# Autodesk Inventor assembly: HTPB14S2M040-K-P3
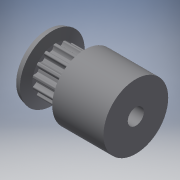
[picture p0: Inventor's stored thumbnail of the model, 180x180]
Saved by Autodesk Inventor 2019 (Build 230136000, 136)
## iProperties
Category: PARTsolutions
Company: MISUMI
Created: 2023-12-23
Part Number: HTPB14S2M040-K-P3
Catalog Web Link: www.cadenas.de
Description: HTPA_ _S2M040, HTPA_ _S2M060, HTPA_ _S2M100, HTPB_ _S2M040, HTPB_ _S2M060, HTPB_ _S2M100, HTPK_ _S2M040, HTPK_ _S2M060, HTPK_ _S2M100, HTPN_ _S2M040, HTPN_ _S2M060, HTPN_ _S2M100, HTPT_ _S2M040, HTPT_ _S2M060, HTPM_ _S2M040, HTPM_ _S2M060, HTPP_ _S2M040, HTPP_ _S2M060, HTPS_ _S2M040, HTPS_ _S2M060, HTPS_ _S2M100-High Torque Timing Pulleys S2M Type
Vendor: MISUMI
Document SubType Name: Assembly
Designer: psAdmin
Manufacturer: MISUMI
Mass: 1.35006 g
Surface Area: 12.4331 cm^2
Volume: 1.35006 cm^3
Density: 1 g/cm^3
Title: HTPB14S2M040-K-P3
Author: Cadenas PARTsolutions
Comments: High Torque Timing Pulleys S2M Type
PSOL_IDENT_0: {$CADENAS_DATA/23d-libs/misumi/metric/51_timing_pulleys/htpm_s2m_asmtab.prj},744 {VTYP=3D},{STYP=ASS
PSOL_IDENT_1: TAB},{NB=HTPB14S2M040-K-P3},{LINA=HTPB14S2M040-K-P3},{NN=HTPA_ _S2M040, HTPA_ _S2M060, HTPA_ _S2M100
PSOL_IDENT_2: , HTPB_ _S2M040, HTPB_ _S2M060, HTPB_ _S2M100, HTPK_ _S2M040, HTPK_ _S2M060, HTPK_ _S2M100, HTPN_ _S
PSOL_IDENT_3: 2M040, HTPN_ _S2M060, HTPN_ _S2M100, HTPT_ _S2M040, HTPT_ _S2M060, HTPM_ _S2M040, HTPM_ _S2M060, HTP
PSOL_IDENT_4: P_ _S2M040, HTPP_ _S2M060, HTPS_ _S2M040, HTPS_ _S2M060, HTPS_ _S2M100},{DATE=13.01.2023 00:39:47},{
PSOL_IDENT_5: GEOMDATE=09.12.2022 07:33:44},{VERSION=},{LINEID=10},{WBVAR=MATP,ST,TNW,PS,SBS,DD,Z,J,Q,R,S,T,ALT1,A
PSOL_IDENT_6: LT2,M,QSC,QFC,QTC,ALT3,K,KSC,KFC,KTC,ALT4,ZM,ZSC,ZFC,ZTC,ALT5,ALT6,ALT7,FC,ALT8,SRG,ALT9,BTC,TL,ALT1
PSOL_IDENT_7: 0,TPC,ALT11,BC,ALT12,SLH,ALT13,BN},{WBNUMERIC=DD,Z,J,Q,R,S,T,QSC,QFC,QTC,K,KSC,KFC,KTC,ZSC,ZFC,ZTC,F
PSOL_IDENT_8: C,SRG,BTC,TL,BC,SLH,BN}  {NB=HTPB14S2M040-K-P3},{LINA=HTPB14S2M040-K-P3},{KT=DUMMY},{PN=HTPB14S2M040
PSOL_IDENT_9: -K-P3},{TYPE=HTPB},{MATP=A2017},{MATPALG= 'A2017','Aluminum Alloy 2000 series','S45CE','1045 Carbon
PSOL_IDENT_10: Steel Equivalent','SUS304','304 Stainless Steel' },{ST=BA},{STALG= 'CA' , 'Clear Anodize', 'BA','Bla
PSOL_IDENT_11: ck Anodize','HAT','Hard Clear Anodize' , 'ENP' , 'Electroless Nickel Plating' },{NT=14},{TNW=S2M040}
PSOL_IDENT_12: ,{TNWALG= 'S2M040', 'S2M060','S2M100' },{BW=4},{PS=K},{PSALG='A','K'},{SBS=P},{SBSALG='H','Round Hol
PSOL_IDENT_13: e','P','Round Hole + Tap'},{SHSA= 'H','Round Hole' },{SHSB='H','Round Hole','P','Round Hole + Tap','
PSOL_IDENT_14: N','New JIS Keywayed Bore + Tap (Standard)','NK','New JIS Keywayed Bore + Tap (width 4.0mm, height 1
PSOL_IDENT_15: .8mm)','C','Old JIS Keywayed Bore + Tap','V','Stepped Hole','F','Stepped Hole (Counterbore holes on
PSOL_IDENT_16: the boss side)' },{SHSK='H','Round Hole','P','Round Hole + Tap'},{SBSPN=-P3},{DD=3.00},{DDALG=[3:4/1
PSOL_IDENT_17: ]},{DDHA=0},{DDHBK=[3:4/1]},{DDPA=0},{DDPBK=[3:4/1]},{DDNA=0},{DDNBK=0},{DDNK=0},{DDCA=0},{DDCBK=0},
PSOL_IDENT_18: {DDVA=0},{DDVF=0},{DDY=0},{DDWB=0},{Z=0},{ZALG=[0]},{ZQRMIN=5},{ZAMAX=0},{ZBMAX=0},{DDZ=3},{J=0.0},{
PSOL_IDENT_19: JALG=[0]},{JMAX=0},{JMIN=2},{JPN=},{QRMAX=0},{QRMIN=5},{WBRMAX=-2.00},{WBQMIN=7},{Q=0},{QALG=[0]},{Q
PSOL_IDENT_20: PN=},{R=0},{RALG=[0]},{S=0.0},{SALG=[0]},{SPN=},{SMAX=3},{T=0.0},{TALG=[0]},{TPN=},{TMAX=6},{A=5},{W=
PSOL_IDENT_21: 9},{L=17},{PD=8.91},{OD=8.40},{D=12},{DALG=12},{DE=12},{F=12},{E=6},{BBK=0.000},{TTK=0.0},{TT=1},{WL=
PSOL_IDENT_22: 17.000},{ALT1=},{ALT1ALG= '','w/o KC90 (Set Screw Angle)','KC90','with KC90 (Set Screw Angle)' },{AN
PSOL_IDENT_23: G=120.000},{ALT1PN=},{ALT2=},{ALT2ALG= '','Not applicable' },{M=N/A},{MALG= 'N/A' },{MFTALG= 'N/A' }
PSOL_IDENT_24: ,{MSALG= 'N/A' },{M3D=0.000},{KDML=0},{ML=0},{MUL=0},{PITCH=0},{QSC=0.0},{QSCALG=0},{QFC=0.0},{QFCAL
PSOL_IDENT_25: G=0},{QTC=0.0},{QTCALG=0},{QPCDMIN=0},{QPCDMINALG=0},{QPCDMAX=8},{ALT2PN=},{ALT3=},{ALT3ALG= '','Not
PSOL_IDENT_26: applicable' },{K=0.0},{KALG=0},{KMIN=4},{KFTMAX=0.0},{KSMAX=0.0},{KSC=0.0},{KSCALG=0},{KFC=0.0},{KF
PSOL_IDENT_27: CALG=0},{KTC=0.0},{KTCALG=0},{KPCDMIN=7},{KPCDMINALG=7},{KPCDMAX=0},{KSCMIN=7.0},{KSCMINALG=7},{ALT3
PSOL_IDENT_28: PN=},{ALT4=},{ALT4ALG= '','Not applicable' },{ALT4MIN=13.5},{ALT4MAX=-4.5},{ZM=N/A},{ZMALG= 'N/A' },
PSOL_IDENT_29: {ZMSALG= 'N/A' },{ZMFTALG= 'N/A' },{ZMDD1=0.0},{ZMDD2=0.0},{ZMHH=0.0},{ZSC=0.0},{ZSCALG=[0]},{ZFC=0.
PSOL_IDENT_30: 0},{ZFCALG=[0]},{ZTC=0.0},{ZTCALG=[0]},{ZPCDMIN=0},{ZPCDMINALG=0},{ZPCDMAX=2},{ALT4PN=},{ALT5=},{ALT
PSOL_IDENT_31: 5ALG= '','Flange Attached','NFC','with NFC (Flange not Attached)' },{ALT5PN=},{ALT6=},{ALT6ALG= '','
PSOL_IDENT_32: Not applicable' },{ALT6PN=},{ALT7=},{ALT7ALG= '','w/o FC (Flange Cut)','FC','with FC (Flange Cut)' }
PSOL_IDENT_33: ,{FC=0.0},{FCALG=0},{FCMIN=9.5},{FCMAX=10.0},{ALT7PN=},{ALT8=},{ALT8ALG= '','Not applicable' },{ALT8
PSOL_IDENT_34: ALGALG=8},{ALT8DD2=0},{ALT8MM=0},{ALT8NN=0},{QC=0},{KC=0},{ZC=0},{SRG=0.0},{SRGALG=[0]},{SRGMAX=0},{
PSOL_IDENT_35: DD2=0.0},{MM=0.00},{NN=0.00},{ALT8PN=},{ALT9ALG= '','Not applicable' },{ALT9=},{BTC9=4},{TL9=1},{BTC=
PSOL_IDENT_36: 0},{BTCALG=[0]},{TL=0.0},{TLALG=[0]},{TLMIN=1.000},{TLMAX=-9.500},{BTCL=0},{BTCD=0},{BTCDALG=6.000},
PSOL_IDENT_37: {ALT9PN=},{WLBCTL=17},{ALT10=},{ALT10ALG= '','w/o TPC (Tapped Hole Dimension)','TPC','with TPC (Tapp
PSOL_IDENT_38: ed Hole Dimension)' },{TPC=N/A},{TPCALG= 'N/A' },{TPCM=3},{ALT10PN=},{ALT11=},{ALT11ALG= '','Not app
PSOL_IDENT_39: licable' },{BC=0.0},{BCALG=0},{BCMIN=6},{BCMAX=7.5},{BCPLANE=12},{M1WBC=12},{ALT11PN=},{ALT12=},{ALT
PSOL_IDENT_40: 12ALG= '','w/o SLH (Set Screw Length)','SLH','with SLH (Set Screw Length)' },{SLH=0},{SLHALG=[0]},{A
PSOL_IDENT_41: LT12PN=},{ALT13=},{ALT13ALG= '', 'Not applicable' },{BN=0.0},{BNALG=0},{BNMIN=8.5},{BNMAX=18},{ALT13
PSOL_IDENT_42: PN=},{AC=M3x3},{M1=3},{M1L=3},{TAP=0.000},{KYY=1.5},{KTT=4.5},{PLANE=0},{PPATH=htpm_s2m/htpa_s2m_asm
PSOL_IDENT_43: tpl.prj}
NB: HTPB14S2M040-K-P3
NN: 0
NT: 14
NBSYN: $PN.
LINA: HTPB14S2M040-K-P3
CATALOG: Misumi
PN: HTPB14S2M040-K-P3
MATP: Aluminum Alloy 2000 series
ST: Black Anodize
TNW: S2M040
BW: 4
PS: K
SBS: Round Hole + Tap
DD: 3
Z: 0
J: 0
Q: 0
R: 0
S: 0
T: 0
A: 5
W: 9
L: 17
PD: 8.91
OD: 8.4
D: 12
F: 12
E: 6
TT: 1
ALT1: w/o KC90 (Set Screw Angle)
ALT2: Not applicable
M: N/A
QSC: 0
QFC: 0
QTC: 0
ALT3: Not applicable
K: 0
KSC: 0
KFC: 0
KTC: 0
ALT4: Not applicable
ZM: N/A
ZMDD1: 0
ZMDD2: 0
ZMHH: 0
ZSC: 0
ZFC: 0
ZTC: 0
ALT5: Flange Attached
ALT6: Not applicable
ALT7: w/o FC (Flange Cut)
FC: 0
ALT8: Not applicable
SRG: 0
DD2: 0
MM: 0
ALT9: Not applicable
BTC: 0
TL: 0
BTCL: 0
BTCD: 0
ALT10: w/o TPC (Tapped Hole Dimension)
TPC: N/A
ALT11: Not applicable
BC: 0
ALT12: w/o SLH (Set Screw Length)
SLH: 0
ALT13: Not applicable
BN: 0
AC: M3x3
SUPPLIER: MISUMI
ARTICLENO: HTPB14S2M040-K-P3
BOMINFO: HTPB14S2M040-K-P3
CREATOR: CADENAS GmbH
## Documents named in this file (3)
- e:\temp\worker_COMMON_2\temp\tmp_7664_2_ImtFj\format_0\HTPB14S2M040-K-P3.iam
- e:\temp\worker_COMMON_2\temp\tmp_7664_2_ImtFj\format_0\HTPB14S2M040-K-P3_a.ipt
- e:\temp\worker_COMMON_2\temp\tmp_7664_2_ImtFj\format_0\SET-SCREW3-3.ipt
## Components (3 placed, 2 different names)
1. HTPB14S2M040-K-P3_a:1 — to_s1_Z@1 <-> CP_Z@2, to_s2_Z@1 <-> CP_Z@3
2. SET-SCREW3-3:1 — to_s1_Z@1 <-> CP_Z@2
3. SET-SCREW3-3:2 — to_s2_Z@1 <-> CP_Z@3
## Relationships (2: Mate 2)
- to_s1_Z@1 <-> CP_Z@2 [Mate]: HTPB14S2M040-K-P3_a:1 ↔ SET-SCREW3-3:1
- to_s2_Z@1 <-> CP_Z@3 [Mate]: HTPB14S2M040-K-P3_a:1 ↔ SET-SCREW3-3:2
